# Autodesk Inventor assembly: USB Head
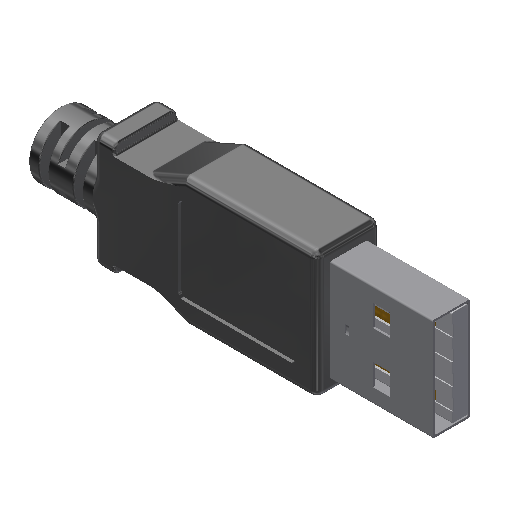
[picture p0: Inventor's stored thumbnail of the model, 512x512]
Saved by Autodesk Inventor 2022 (Build 260153000, 153)
## iProperties
Created: 2021-05-12
Part Number: USB Head
Document SubType Name: Assembly
Designer: bayua
Author: bayua
## Documents named in this file (4)
- C:\Users\ferna\Downloads\usb-head-18.snapshot.1\USB Head.iam
- C:\Users\ferna\Downloads\usb-head-18.snapshot.1\USB-Housing.ipt
- C:\Users\ferna\Downloads\usb-head-18.snapshot.1\USB-Connector1.ipt
- C:\Users\ferna\Downloads\usb-head-18.snapshot.1\USB-Recaptacles1.ipt
## Components (3 placed, 3 different names)
1. USB-Housing:1 — Mate:1, Mate:2, Mate:3
2. USB-Connector1:1 — Mate:1, Mate:2, Mate:3, Mate:4, Mate:5, Mate:6
3. USB-Recaptacles1:1 — Mate:4, Mate:5, Mate:6
## Relationships (6: Mate 6)
- Mate:1: USB-Housing:1 ↔ USB-Connector1:1
- Mate:2: USB-Housing:1 ↔ USB-Connector1:1
- Mate:3: USB-Housing:1 ↔ USB-Connector1:1
- Mate:4: USB-Connector1:1 ↔ USB-Recaptacles1:1
- Mate:5: USB-Connector1:1 ↔ USB-Recaptacles1:1
- Mate:6: USB-Connector1:1 ↔ USB-Recaptacles1:1
